# Autodesk Inventor assembly: gun 3_ЗЕРКАЛО
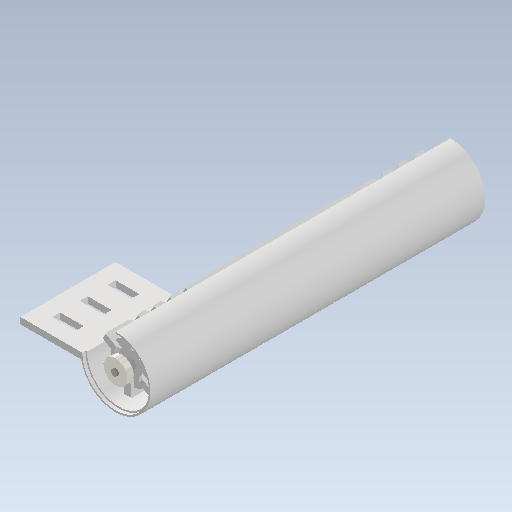
[picture p0: Inventor's stored thumbnail of the model, 512x512]
Saved by Autodesk Inventor 2020.1 (Build 241239000, 239)
## iProperties
Created: 2022-04-02
Part Number: gun 3_ЗЕРКАЛО
Document SubType Name: Assembly
Designer: User
Author: User
## Documents named in this file (6)
- D:\GitHub\TANK\3D-turret\gun 3_ЗЕРКАЛО.iam
- D:\GitHub\TANK\3D-turret\barrel_holder_ЗЕРКАЛО.ipt
- D:\GitHub\TANK\3D-turret\trunk_ЗЕРКАЛО.ipt
- D:\GitHub\TANK\3D-turret\ось пушки 3_ЗЕРКАЛО.ipt
- D:\GitHub\TANK\3D-turret\подшипник_ЗЕРКАЛО.ipt
- D:\GitHub\TANK\3D-turret\кожух пушки_ЗЕРКАЛО.ipt
## Components (12 placed, 5 different names)
1. barrel_holder_ЗЕРКАЛО:1 — Жесткий:1, Жесткий:3
2. barrel_holder_ЗЕРКАЛО:2 — Жесткий:2
3. ось пушки 3_ЗЕРКАЛО:1 — Жесткий:3, Жесткий:4, Жесткий:5
4. подшипник_ЗЕРКАЛО:1 — Совмещение:1, Жесткий:4
5. подшипник_ЗЕРКАЛО:2 — Жесткий:5
6. кожух пушки_ЗЕРКАЛО:1 — Совмещение:1
7. trunk_ЗЕРКАЛО:1 — Жесткий:1
8. trunk_ЗЕРКАЛО:2
9. trunk_ЗЕРКАЛО:3 — Жесткий:2
10. trunk_ЗЕРКАЛО:4
11. trunk_ЗЕРКАЛО:5
12. trunk_ЗЕРКАЛО:6
## Component patterns: (6 elements, first: trunk_ЗЕРКАЛО:1)
## Relationships (6: WeldJoint 5, Mate 1)
- Совмещение:1 [Mate]: подшипник_ЗЕРКАЛО:1 ↔ кожух пушки_ЗЕРКАЛО:1
- Жесткий:1 [WeldJoint]: barrel_holder_ЗЕРКАЛО:1 ↔ trunk_ЗЕРКАЛО:1
- Жесткий:3 [WeldJoint]: barrel_holder_ЗЕРКАЛО:1 ↔ ось пушки 3_ЗЕРКАЛО:1
- Жесткий:4 [WeldJoint]: ось пушки 3_ЗЕРКАЛО:1 ↔ подшипник_ЗЕРКАЛО:1
- Жесткий:5 [WeldJoint]: ось пушки 3_ЗЕРКАЛО:1 ↔ подшипник_ЗЕРКАЛО:2
- Жесткий:2 [WeldJoint]: barrel_holder_ЗЕРКАЛО:2 ↔ trunk_ЗЕРКАЛО:3
